# Autodesk Inventor assembly: ZMotor
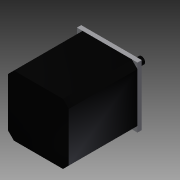
[picture p0: Inventor's stored thumbnail of the model, 180x180]
Saved by Autodesk Inventor 2015 (Build 190159000, 159)
## iProperties
Created: 2014-08-12
Part Number: ZMotor
Document SubType Name: Assembly
Designer: Jack
Author: Jack
## Documents named in this file (3)
- C:\Users\t_clevj\ownCloud\CoreXY\InventorModel\ZAxis\ZMotor.iam
- C:\Users\t_clevj\ownCloud\CoreXY\InventorModel\Electronics\Motors\StepperMotorNema17.ipt
- C:\Users\t_clevj\ownCloud\CoreXY\InventorModel\ZAxis\ZMotorMount.ipt
## Components (2 placed, 2 different names)
1. StepperMotorNema17:1 — Mate:1, Mate:2, Angle:1
2. ZMotorMount:1 — Mate:1, Mate:2, Angle:1
## Relationships (3: Mate 2, Angle 1)
- Mate:1: StepperMotorNema17:1 ↔ ZMotorMount:1
- Mate:2: StepperMotorNema17:1 ↔ ZMotorMount:1
- Angle:1 (0 deg): StepperMotorNema17:1 ↔ ZMotorMount:1
